# Autodesk Inventor assembly: humidity_sensor
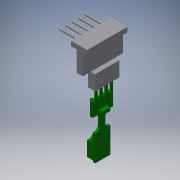
[picture p0: Inventor's stored thumbnail of the model, 180x180]
Saved by Autodesk Inventor 2017.2 (Build 212233000, 233)
## iProperties
Created: 2017-10-12
Part Number: humidity_sensor
Document SubType Name: Assembly
Designer: Nic
Author: Nic
## Documents named in this file (3)
- C:\Users\Nic\Documents\iDripper\humidity_sensor.iam
- C:\Users\Nic\Documents\HumiditySensingRig\humidity_sensor_part.ipt
- C:\Users\Nic\Documents\iDripper\humidity_sensor_mount.ipt
## Components (2 placed, 2 different names)
1. humidity_sensor_part:1 — Insert:1, Insert:2
2. humidity_sensor_mount:1 — Insert:1, Insert:2
## Relationships (2: Insert 2)
- Insert:1: humidity_sensor_part:1 ↔ humidity_sensor_mount:1
- Insert:2: humidity_sensor_part:1 ↔ humidity_sensor_mount:1
